# Autodesk Inventor assembly: Motor Mount with Motor
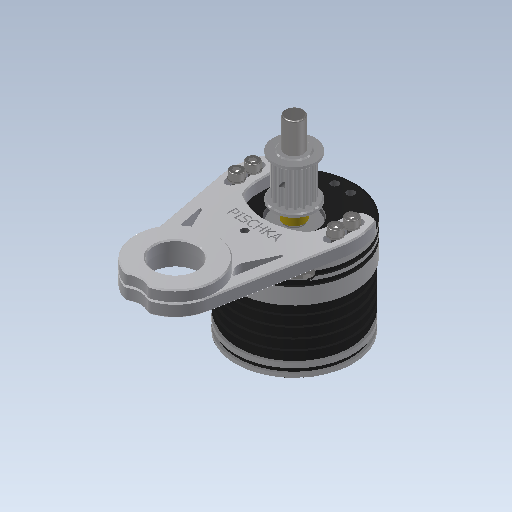
[picture p0: Inventor's stored thumbnail of the model, 512x512]
Saved by Autodesk Inventor 2020.1 (Build 241239000, 239)
## iProperties
Created: 2019-03-01
Part Number: Motor Mount with Motor
Document SubType Name: Assembly
Designer: Petar
Mass: 37.7633 g
Surface Area: 102.459 cm^2
Volume: 12.7696 cm^3
Density: 2.95729 g/cm^3
Author: Petar
## Documents named in this file (9)
- D:\OMG\E-Board\CAD\Inventor\Mechanical Components\Assemblies\Motor Mount (Left-225-ABS) with Motor - Kopie.iam
- D:\OMG\E-Board\CAD\Inventor\Mechanical Components\Motor Mount\Ring Mount\Mount Ring - ABS.ipt
- D:\OMG\E-Board\CAD\Inventor\Electric Motor\Turnigy SK8 5045.iam
- D:\OMG\E-Board\CAD\Inventor\Mechanical Components\Motor Mount\Holder Mount\Motor Holder v3 - 225 - ABS.ipt
- D:\OMG\E-Board\CAD\Inventor\Mechanical Components\Assemblies\Motor Mount (Left-225-ABS) with Motor - Kopie\Design Accelerator\Bolted Connection1.iam
- D:\OMG\E-Board\CAD\Inventor\Mechanical Components\Assemblies\Motor Mount (Left-225-ABS) with Motor - Kopie\Design Accelerator\Bolted Connection2.iam
- D:\OMG\E-Board\CAD\Inventor\Mechanical Components\Assemblies\Motor Mount (Left-225-ABS) with Motor - Kopie\Design Accelerator\Bolted Connection3.iam
- D:\OMG\E-Board\CAD\Inventor\Mechanical Components\Assemblies\Motor Mount (Left-225-ABS) with Motor - Kopie\Design Accelerator\Bolted Connection4.iam
- D:\OMG\E-Board\CAD\Inventor\Mechanical Components\Assemblies\Motor Mount with Motor\AIP\FEA\ct0fs66e9.fres
## Components (7 placed, 4 different names)
1. Mount Ring - ABS:1 — Rigid:1
2. Motor Holder v3 - 225 - ABS:1 — Rigid:1, Rigid:2, Mate:1, Mate:3, Mate:5, Mate:7
3. Turnigy SK8 5045:1 [sub-assembly] — Rigid:2, Mate:2, Mate:4, Mate:6, Mate:8
4. Bolted Connection:1 [sub-assembly] — Mate:1, Mate:2
5. Bolted Connection:2 [sub-assembly] — Mate:3, Mate:4
6. Bolted Connection:3 [sub-assembly] — Mate:5, Mate:6
7. Bolted Connection:4 [sub-assembly] — Mate:7, Mate:8
## Relationships (10: Mate 8, WeldJoint 2)
- Rigid:1 [WeldJoint]: Mount Ring - ABS:1 ↔ Motor Holder v3 - 225 - ABS:1
- Rigid:2 [WeldJoint]: Motor Holder v3 - 225 - ABS:1 ↔ Turnigy SK8 5045:1
- Mate:1: Motor Holder v3 - 225 - ABS:1 ↔ Bolted Connection:1
- Mate:2: Turnigy SK8 5045:1 ↔ Bolted Connection:1
- Mate:3: Motor Holder v3 - 225 - ABS:1 ↔ Bolted Connection:2
- Mate:4: Turnigy SK8 5045:1 ↔ Bolted Connection:2
- Mate:5: Motor Holder v3 - 225 - ABS:1 ↔ Bolted Connection:3
- Mate:6: Turnigy SK8 5045:1 ↔ Bolted Connection:3
- Mate:7: Motor Holder v3 - 225 - ABS:1 ↔ Bolted Connection:4
- Mate:8: Turnigy SK8 5045:1 ↔ Bolted Connection:4
